# Autodesk Inventor assembly: stopper_new
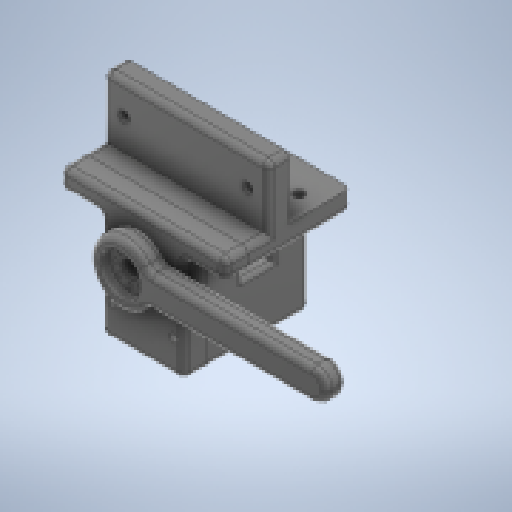
[picture p0: Inventor's stored thumbnail of the model, 512x512]
Saved by Autodesk Inventor 2026.2 (Build 302298010, 298A)
## iProperties
Created: 2026-05-22
Part Number: stopper_new
Document SubType Name: Assembly
Designer: chris
Author: chris
## Documents named in this file (6)
- C:\Users\chanh\내 드라이브\교과공부\2026년 1학기 (4학년 1학기)\01창의제품설계\UMMA_CAD\02하체\Stopper\stopper.iam
- C:\Users\chanh\내 드라이브\교과공부\2026년 1학기 (4학년 1학기)\01창의제품설계\UMMA_CAD\02하체\Stopper\stopper_motor_bracket.ipt
- C:\Users\chanh\내 드라이브\교과공부\2026년 1학기 (4학년 1학기)\01창의제품설계\UMMA_CAD\02하체\Stopper\stopper_motor_bracket_cover.ipt
- C:\Users\chanh\내 드라이브\교과공부\2026년 1학기 (4학년 1학기)\01창의제품설계\UMMA_CAD\02하체\Stopper\stopper_rod.ipt
- C:\Users\chanh\내 드라이브\교과공부\2026년 1학기 (4학년 1학기)\01창의제품설계\UMMA_CAD\02하체\Stopper\HTD-45H.ipt
- C:\Users\chanh\내 드라이브\교과공부\2026년 1학기 (4학년 1학기)\01창의제품설계\UMMA_CAD\02하체\Stopper\Top Horn.ipt
## Components (5 placed, 5 different names)
1. stopper_motor_bracket:1 — Flush:1, Flush:2, Mate:1, Mate:2, Flush:3, Flush:8, Mate:4, Flush:9, Mate:6
2. stopper_motor_bracket_cover:1 — Flush:1, Flush:2, Mate:6
3. stopper_rod:1 — Rigid:1
4. HTD-45H:1 — Flush:8, Mate:4, Flush:9, Rotational:1
5. Top Horn:1 — Rigid:1, Rotational:1
## Relationships (11: Flush 5, Mate 4, WeldJoint 1, RevoluteJoint 1)
- Flush:1: stopper_motor_bracket:1 ↔ stopper_motor_bracket_cover:1
- Flush:2: stopper_motor_bracket:1 ↔ stopper_motor_bracket_cover:1
- Mate:1: stopper_motor_bracket:1
- Mate:2: stopper_motor_bracket:1
- Flush:3: stopper_motor_bracket:1
- Flush:8: stopper_motor_bracket:1 ↔ HTD-45H:1
- Mate:4: stopper_motor_bracket:1 ↔ HTD-45H:1
- Flush:9: stopper_motor_bracket:1 ↔ HTD-45H:1
- Mate:6: stopper_motor_bracket:1 ↔ stopper_motor_bracket_cover:1
- Rigid:1 [WeldJoint]: stopper_rod:1 ↔ Top Horn:1
- Rotational:1 [RevoluteJoint]: HTD-45H:1 ↔ Top Horn:1
